# Autodesk Inventor assembly: Eje_Engrane-llanta
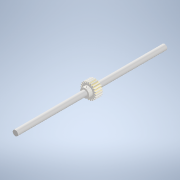
[picture p0: Inventor's stored thumbnail of the model, 180x180]
Saved by Autodesk Inventor 2021 (Build 250183000, 183)
## iProperties
Created: 2021-02-07
Part Number: Eje_Engrane-llanta
Document SubType Name: Assembly
Designer: rotje
Author: rotje
## Documents named in this file (3)
- C:\Users\rotje\Documents\Inventor\MSF\Eje_Engrane-llanta.iam
- C:\Users\rotje\Documents\Inventor\MSF\Eje_Engranes_llanta.ipt
- C:\Users\rotje\Documents\Inventor\MSF\Engranaje recto_20_Dientes.ipt
## Components (2 placed, 2 different names)
1. Eje_Engranes_llanta:1 — Insertar:1
2. Engranaje recto1:1 — Insertar:1
## Relationships (1: Insert 1)
- Insertar:1: Eje_Engranes_llanta:1 ↔ Engranaje recto1:1
